# Autodesk Inventor assembly: Bed Assembly
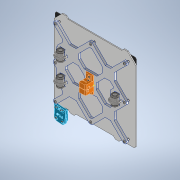
[picture p0: Inventor's stored thumbnail of the model, 180x180]
Saved by Autodesk Inventor 2021 (Build 250183000, 183)
## iProperties
Created: 2019-09-16
Part Number: Bed Assembly
Document SubType Name: Assembly
Designer: pepd9
Author: pepd9
## Documents named in this file (20)
- D:\Designs\MK3PRO P1\BED ASSEMBLY\Bed Assembly.iam
- D:\Designs\MK3PRO P1\BED ASSEMBLY\FROG.ipt
- D:\Designs\MK3PRO P1\BED ASSEMBLY\19mm ID UBOLT.ipt
- D:\Designs\MK3PRO P1\COMPONENTS\LM10UU.ipt
- D:\Designs\MK3PRO P1\COMPONENTS\90494A029_LOW-STRENGTH STEEL THIN HEX NUT.ipt
- D:\Designs\MK3PRO P1\COMPONENTS\BHCS M3_6.ipt
- D:\Designs\MK3PRO P1\COMPONENTS\6x6x3t spacer.ipt
- D:\Designs\MK3PRO P1\BED ASSEMBLY\MK52 Bed.ipt
- D:\Designs\MK3PRO P1\COMPONENTS\FHCS - M3x5.ipt
- D:\Designs\MK3PRO P1\COMPONENTS\M3 Lockwasher.ipt
- D:\Designs\MK3PRO P1\BED ASSEMBLY\SS Sheet.ipt
- D:\Designs\MK3PRO P1\BED ASSEMBLY\heatbed-cable-cover top.ipt
- D:\Designs\MK3PRO P1\BED ASSEMBLY\heatbed-cable-cover bottom.ipt
- D:\Designs\MK3PRO P1\BED ASSEMBLY\y-belt-holder.ipt
- D:\Designs\MK3PRO P1\BED ASSEMBLY\y-belt-tensioner.ipt
- D:\Designs\MK3PRO P1\COMPONENTS\SHCS_M3_30.ipt
- D:\Designs\MK3PRO P1\COMPONENTS\SHCS_M3_8.ipt
- D:\Designs\MK3PRO P1\COMPONENTS\M3 Nut.ipt
- D:\Designs\MK3PRO P1\COMPONENTS\M3 Washer.ipt
- D:\Designs\MK3PRO P1\COMPONENTS\SHCS_M3_12.ipt
## Components (72 placed, 19 different names)
1. FROG:1 — Mate:1, Mate:2, Flush:1, Mate:3, Mate:4, Mate:5, Mate:6, Mate:7, Mate:8, Tangent:1, Tangent:2, Tangent:3, Mate:12, Mate:13, Mate:14, Mate:15, Mate:16, Mate:17, Mate:18, Mate:19, Mate:20, Mate:27, Mate:28, Mate:29, Mate:30, Mate:31, Mate:32, Mate:33, Mate:34, Mate:35, Mate:45, Mate:46, Mate:47, Mate:48, Mate:49, Mate:50, Mate:51, Mate:53, Mate:102, Mate:109, Mate:110, Mate:170, Angle:5
2. 19mm ID UBOLT:1 — Mate:5, Mate:6, Mate:10, Mate:25, Mate:26
3. 19mm ID UBOLT:2 — Mate:7, Mate:8, Mate:11, Mate:21, Mate:22
4. 19mm ID UBOLT:3 — Mate:3, Mate:4, Mate:9, Mate:23, Mate:24
5. LM10UU:1 — Mate:11, Tangent:2, Mate:14
6. LM10UU:2 — Mate:10, Tangent:3, Mate:12
7. LM10UU:3 — Mate:9, Tangent:1, Mate:13
8. 90494A029_LOW-STRENGTH STEEL THIN HEX NUT:1 — Mate:17, Mate:25
9. 90494A029_LOW-STRENGTH STEEL THIN HEX NUT:2 — Mate:18, Mate:26
10. 90494A029_LOW-STRENGTH STEEL THIN HEX NUT:3 — Mate:16, Mate:23
11. 90494A029_LOW-STRENGTH STEEL THIN HEX NUT:4 — Mate:15, Mate:24
12. 90494A029_LOW-STRENGTH STEEL THIN HEX NUT:5 — Mate:20, Mate:21
13. 90494A029_LOW-STRENGTH STEEL THIN HEX NUT:6 — Mate:19, Mate:22
14. BHCS M3_6:1 — Mate:29, Mate:54
15. BHCS M3_6:2 — Mate:28, Mate:55
16. BHCS M3_6:3 — Mate:27, Mate:56
17. BHCS M3_6:4 — Mate:31
18. BHCS M3_6:5 — Mate:30
19. BHCS M3_6:6 — Mate:32
20. BHCS M3_6:7 — Mate:35, Mate:58
21. BHCS M3_6:8 — Mate:34, Mate:59
22. BHCS M3_6:9 — Mate:33, Mate:61
23. 6x6x3t spacer:1 — Mate:47, Mate:56, Mate:98
24. 6x6x3t spacer:2 — Mate:46, Mate:58, Mate:99
25. 6x6x3t spacer:3 — Mate:45, Mate:100
26. 6x6x3t spacer:4 — Mate:49
27. 6x6x3t spacer:5 — Mate:48, Mate:59
28. 6x6x3t spacer:6 — Mate:50, Mate:55
29. 6x6x3t spacer:7 — Mate:51, Mate:61
30. 6x6x3t spacer:9 — Mate:53, Mate:54
31. MK52 Bed:1 — Mate:62, Mate:63, Mate:64, Mate:65, Mate:66, Mate:67, Mate:68, Mate:69, Mate:70, Mate:71, Mate:72, Mate:73, Mate:74, Mate:75, Mate:76, Mate:77, Mate:78, Mate:79, Mate:80, Mate:82, Mate:83, Mate:84, Mate:85, Mate:86, Mate:87, Mate:88, Mate:89, Mate:101, Angle:1, Mate:130, Mate:132, Mate:133, Mate:134, Mate:135, Mate:140, Mate:141, Mate:152
32. FHCS - M3x5:1 — Mate:62, Mate:63, Mate:97, Mate:98
33. FHCS - M3x5:2 — Mate:64, Mate:72, Mate:94
34. FHCS - M3x5:3 — Mate:65, Mate:73, Mate:96
35. FHCS - M3x5:4 — Mate:66, Mate:74, Mate:95, Mate:103
36. FHCS - M3x5:5 — Mate:67, Mate:75, Mate:93
37. FHCS - M3x5:6 — Mate:68, Mate:76, Mate:91
38. FHCS - M3x5:7 — Mate:69, Mate:77, Mate:90, Mate:99
39. FHCS - M3x5:8 — Mate:70, Mate:78, Mate:92
40. FHCS - M3x5:9 — Mate:71, Mate:79, Mate:81
41. M3 Lockwasher:1 — Mate:84, Mate:95
42. M3 Lockwasher:2 — Mate:83, Mate:90
43. M3 Lockwasher:3 — Mate:82, Mate:92
44. M3 Lockwasher:4 — Mate:80, Mate:81
45. M3 Lockwasher:5 — Mate:85, Mate:93
46. M3 Lockwasher:6 — Mate:86, Mate:91, Mate:100
47. M3 Lockwasher:7 — Mate:88, Mate:94
48. M3 Lockwasher:8 — Mate:89, Mate:97
49. M3 Lockwasher:9 — Mate:87, Mate:96
50. SS Sheet:1 — Mate:101
51. 6x6x3t spacer:10 — Mate:102, Mate:103
52. heatbed-cable-cover top:1 — Mate:106, Angle:1, Mate:130, Mate:152, Mate:153, Mate:154, Mate:155, Mate:156
53. heatbed-cable-cover bottom:1 — Mate:106, Mate:157, Mate:159, Mate:160, Mate:162, Angle:2
54. y-belt-holder:1 — Mate:110, Mate:114, Mate:115, Mate:116, Mate:170, Angle:5
55. y-belt-tensioner:1 — Mate:109, Mate:112, Mate:113, Mate:118
56. SHCS_M3_30:1 — Mate:112, Mate:113, Mate:114
57. SHCS_M3_8:1 — Mate:115, Mate:116
58. SHCS_M3_8:2 — Mate:118
59. SHCS_M3_8:5 — Mate:133, Mate:137, Mate:138, Mate:142, Mate:146, Mate:150
60. SHCS_M3_8:6 — Mate:132, Mate:136, Mate:139, Mate:143, Mate:147, Mate:151
61. M3 Washer:1 — Mate:134, Mate:136, Mate:139
62. M3 Washer:2 — Mate:135, Mate:137, Mate:138
63. M3 Washer:3 — Mate:140, Mate:142, Mate:144
64. M3 Washer:4 — Mate:141, Mate:143, Mate:145
65. M3 Lockwasher:10 — Mate:145, Mate:147, Mate:149
66. M3 Lockwasher:11 — Mate:144, Mate:146, Mate:148
67. M3 Nut:3 — Mate:148, Mate:150
68. M3 Nut:4 — Mate:149, Mate:151, Angle:2
69. SHCS_M3_12:1 — Mate:154, Mate:156, Mate:158
70. SHCS_M3_12:2 — Mate:153, Mate:155, Mate:161
71. M3 Nut:5 — Mate:157, Mate:158, Mate:159
72. M3 Nut:6 — Mate:160, Mate:161, Mate:162
## Relationships (140: Mate 133, Tangent 3, Angle 3, Flush 1)
- Mate:1 (-3.175 mm): FROG:1
- Mate:2 (-113.5 mm): FROG:1
- Flush:1 (-114.5 mm): FROG:1
- Mate:3: FROG:1 ↔ 19mm ID UBOLT:3
- Mate:4: FROG:1 ↔ 19mm ID UBOLT:3
- Mate:5: FROG:1 ↔ 19mm ID UBOLT:1
- Mate:6: FROG:1 ↔ 19mm ID UBOLT:1
- Mate:7: FROG:1 ↔ 19mm ID UBOLT:2
- Mate:8: FROG:1 ↔ 19mm ID UBOLT:2
- Mate:9: 19mm ID UBOLT:3 ↔ LM10UU:3
- Mate:10: 19mm ID UBOLT:1 ↔ LM10UU:2
- Mate:11: 19mm ID UBOLT:2 ↔ LM10UU:1
- Tangent:1: FROG:1 ↔ LM10UU:3
- Tangent:2: FROG:1 ↔ LM10UU:1
- Tangent:3: FROG:1 ↔ LM10UU:2
- Mate:12 (1.5 mm): FROG:1 ↔ LM10UU:2
- Mate:13 (1.5 mm): FROG:1 ↔ LM10UU:3
- Mate:14 (1.5 mm): FROG:1 ↔ LM10UU:1
- Mate:15: FROG:1 ↔ 90494A029_LOW-STRENGTH STEEL THIN HEX NUT:4
- Mate:16: FROG:1 ↔ 90494A029_LOW-STRENGTH STEEL THIN HEX NUT:3
- Mate:17: FROG:1 ↔ 90494A029_LOW-STRENGTH STEEL THIN HEX NUT:1
- Mate:18: FROG:1 ↔ 90494A029_LOW-STRENGTH STEEL THIN HEX NUT:2
- Mate:19: FROG:1 ↔ 90494A029_LOW-STRENGTH STEEL THIN HEX NUT:6
- Mate:20: FROG:1 ↔ 90494A029_LOW-STRENGTH STEEL THIN HEX NUT:5
- Mate:21: 19mm ID UBOLT:2 ↔ 90494A029_LOW-STRENGTH STEEL THIN HEX NUT:5
- Mate:22: 19mm ID UBOLT:2 ↔ 90494A029_LOW-STRENGTH STEEL THIN HEX NUT:6
- Mate:23: 19mm ID UBOLT:3 ↔ 90494A029_LOW-STRENGTH STEEL THIN HEX NUT:3
- Mate:24: 19mm ID UBOLT:3 ↔ 90494A029_LOW-STRENGTH STEEL THIN HEX NUT:4
- Mate:25: 19mm ID UBOLT:1 ↔ 90494A029_LOW-STRENGTH STEEL THIN HEX NUT:1
- Mate:26: 19mm ID UBOLT:1 ↔ 90494A029_LOW-STRENGTH STEEL THIN HEX NUT:2
- Mate:27: FROG:1 ↔ BHCS M3_6:3
- Mate:28: FROG:1 ↔ BHCS M3_6:2
- Mate:29: FROG:1 ↔ BHCS M3_6:1
- Mate:30: FROG:1 ↔ BHCS M3_6:5
- Mate:31: FROG:1 ↔ BHCS M3_6:4
- Mate:32: FROG:1 ↔ BHCS M3_6:6
- Mate:33: FROG:1 ↔ BHCS M3_6:9
- Mate:34: FROG:1 ↔ BHCS M3_6:8
- Mate:35: FROG:1 ↔ BHCS M3_6:7
- Mate:45: FROG:1 ↔ 6x6x3t spacer:3
- Mate:46: FROG:1 ↔ 6x6x3t spacer:2
- Mate:47: FROG:1 ↔ 6x6x3t spacer:1
- Mate:48: FROG:1 ↔ 6x6x3t spacer:5
- Mate:49: FROG:1 ↔ 6x6x3t spacer:4
- Mate:50: FROG:1 ↔ 6x6x3t spacer:6
- Mate:51: FROG:1 ↔ 6x6x3t spacer:7
- Mate:53: FROG:1 ↔ 6x6x3t spacer:9
- Mate:54: BHCS M3_6:1 ↔ 6x6x3t spacer:9
- Mate:55: BHCS M3_6:2 ↔ 6x6x3t spacer:6
- Mate:56: BHCS M3_6:3 ↔ 6x6x3t spacer:1
- Mate:58: BHCS M3_6:7 ↔ 6x6x3t spacer:2
- Mate:59: BHCS M3_6:8 ↔ 6x6x3t spacer:5
- Mate:61: BHCS M3_6:9 ↔ 6x6x3t spacer:7
- Mate:62: MK52 Bed:1 ↔ FHCS - M3x5:1
- Mate:63: MK52 Bed:1 ↔ FHCS - M3x5:1
- Mate:64: MK52 Bed:1 ↔ FHCS - M3x5:2
- Mate:65: MK52 Bed:1 ↔ FHCS - M3x5:3
- Mate:66: MK52 Bed:1 ↔ FHCS - M3x5:4
- Mate:67: MK52 Bed:1 ↔ FHCS - M3x5:5
- Mate:68: MK52 Bed:1 ↔ FHCS - M3x5:6
- Mate:69: MK52 Bed:1 ↔ FHCS - M3x5:7
- Mate:70: MK52 Bed:1 ↔ FHCS - M3x5:8
- Mate:71: MK52 Bed:1 ↔ FHCS - M3x5:9
- Mate:72: MK52 Bed:1 ↔ FHCS - M3x5:2
- Mate:73: MK52 Bed:1 ↔ FHCS - M3x5:3
- Mate:74: MK52 Bed:1 ↔ FHCS - M3x5:4
- Mate:75: MK52 Bed:1 ↔ FHCS - M3x5:5
- Mate:76: MK52 Bed:1 ↔ FHCS - M3x5:6
- Mate:77: MK52 Bed:1 ↔ FHCS - M3x5:7
- Mate:78: MK52 Bed:1 ↔ FHCS - M3x5:8
- Mate:79: MK52 Bed:1 ↔ FHCS - M3x5:9
- Mate:80: MK52 Bed:1 ↔ M3 Lockwasher:4
- Mate:81: FHCS - M3x5:9 ↔ M3 Lockwasher:4
- Mate:82: MK52 Bed:1 ↔ M3 Lockwasher:3
- Mate:83: MK52 Bed:1 ↔ M3 Lockwasher:2
- Mate:84: MK52 Bed:1 ↔ M3 Lockwasher:1
- Mate:85: MK52 Bed:1 ↔ M3 Lockwasher:5
- Mate:86: MK52 Bed:1 ↔ M3 Lockwasher:6
- Mate:87: MK52 Bed:1 ↔ M3 Lockwasher:9
- Mate:88: MK52 Bed:1 ↔ M3 Lockwasher:7
- Mate:89: MK52 Bed:1 ↔ M3 Lockwasher:8
- Mate:90: FHCS - M3x5:7 ↔ M3 Lockwasher:2
- Mate:91: FHCS - M3x5:6 ↔ M3 Lockwasher:6
- Mate:92: FHCS - M3x5:8 ↔ M3 Lockwasher:3
- Mate:93: FHCS - M3x5:5 ↔ M3 Lockwasher:5
- Mate:94: FHCS - M3x5:2 ↔ M3 Lockwasher:7
- Mate:95: FHCS - M3x5:4 ↔ M3 Lockwasher:1
- Mate:96: FHCS - M3x5:3 ↔ M3 Lockwasher:9
- Mate:97: FHCS - M3x5:1 ↔ M3 Lockwasher:8
- Mate:98: 6x6x3t spacer:1 ↔ FHCS - M3x5:1
- Mate:99: 6x6x3t spacer:2 ↔ FHCS - M3x5:7
- Mate:100: 6x6x3t spacer:3 ↔ M3 Lockwasher:6
- Mate:101: MK52 Bed:1 ↔ SS Sheet:1
- Mate:102: FROG:1 ↔ 6x6x3t spacer:10
- Mate:103: FHCS - M3x5:4 ↔ 6x6x3t spacer:10
- Mate:106: heatbed-cable-cover top:1 ↔ heatbed-cable-cover bottom:1
- Mate:109: FROG:1 ↔ y-belt-tensioner:1
- Mate:110: FROG:1 ↔ y-belt-holder:1
- Mate:112: y-belt-tensioner:1 ↔ SHCS_M3_30:1
- Mate:113: y-belt-tensioner:1 ↔ SHCS_M3_30:1
- Mate:114: y-belt-holder:1 ↔ SHCS_M3_30:1
- Mate:115: y-belt-holder:1 ↔ SHCS_M3_8:1
- Mate:116: y-belt-holder:1 ↔ SHCS_M3_8:1
- Mate:118: y-belt-tensioner:1 ↔ SHCS_M3_8:2
- Angle:1 (180 deg): MK52 Bed:1 ↔ heatbed-cable-cover top:1
- Mate:130: MK52 Bed:1 ↔ heatbed-cable-cover top:1
- Mate:132: MK52 Bed:1 ↔ SHCS_M3_8:6
- Mate:133: MK52 Bed:1 ↔ SHCS_M3_8:5
- Mate:134: MK52 Bed:1 ↔ M3 Washer:1
- Mate:135: MK52 Bed:1 ↔ M3 Washer:2
- Mate:136: SHCS_M3_8:6 ↔ M3 Washer:1
- Mate:137: SHCS_M3_8:5 ↔ M3 Washer:2
- Mate:138: SHCS_M3_8:5 ↔ M3 Washer:2
- Mate:139: SHCS_M3_8:6 ↔ M3 Washer:1
- Mate:140: MK52 Bed:1 ↔ M3 Washer:3
- Mate:141: MK52 Bed:1 ↔ M3 Washer:4
- Mate:142: SHCS_M3_8:5 ↔ M3 Washer:3
- Mate:143: SHCS_M3_8:6 ↔ M3 Washer:4
- Mate:144: M3 Washer:3 ↔ M3 Lockwasher:11
- Mate:145: M3 Washer:4 ↔ M3 Lockwasher:10
- Mate:146: SHCS_M3_8:5 ↔ M3 Lockwasher:11
- Mate:147: SHCS_M3_8:6 ↔ M3 Lockwasher:10
- Mate:148: M3 Lockwasher:11 ↔ M3 Nut:3
- Mate:149: M3 Lockwasher:10 ↔ M3 Nut:4
- Mate:150: SHCS_M3_8:5 ↔ M3 Nut:3
- Mate:151: SHCS_M3_8:6 ↔ M3 Nut:4
- Mate:152: MK52 Bed:1 ↔ heatbed-cable-cover top:1
- Mate:153: heatbed-cable-cover top:1 ↔ SHCS_M3_12:2
- Mate:154: heatbed-cable-cover top:1 ↔ SHCS_M3_12:1
- Mate:155: heatbed-cable-cover top:1 ↔ SHCS_M3_12:2
- Mate:156: heatbed-cable-cover top:1 ↔ SHCS_M3_12:1
- Mate:157: heatbed-cable-cover bottom:1 ↔ M3 Nut:5
- Mate:158: SHCS_M3_12:1 ↔ M3 Nut:5
- Mate:159: heatbed-cable-cover bottom:1 ↔ M3 Nut:5
- Mate:160: heatbed-cable-cover bottom:1 ↔ M3 Nut:6
- Mate:161: SHCS_M3_12:2 ↔ M3 Nut:6
- Mate:162: heatbed-cable-cover bottom:1 ↔ M3 Nut:6
- Angle:2 (0 deg): heatbed-cable-cover bottom:1 ↔ M3 Nut:4
- Mate:170: FROG:1 ↔ y-belt-holder:1
- Angle:5 (0 deg): FROG:1 ↔ y-belt-holder:1
